# Autodesk Inventor assembly: ThrusterAssembly
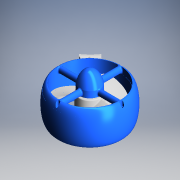
[picture p0: Inventor's stored thumbnail of the model, 180x180]
Saved by Autodesk Inventor 2016 (Build 200138000, 138)
## iProperties
Created: 2016-02-28
Part Number: ThrusterAssembly
Document SubType Name: Assembly
Designer: Willis
Author: Willis
## Documents named in this file (7)
- C:\Users\Willis\Desktop\ROV2015\Thruster Beta\ThrusterAssembly.iam
- C:\Users\Willis\Desktop\ROV2015\Thruster Beta\Body.ipt
- C:\Users\Willis\Desktop\ROV2015\Thruster Beta\Cap.ipt
- C:\Users\Willis\Desktop\ROV2015\Thruster Beta\BrushlessInner.ipt
- C:\Users\Willis\Desktop\ROV2015\Thruster Beta\BrushlessOuter.ipt
- C:\Users\Willis\Desktop\ROV2015\Thruster Beta\Prop_Mk2.ipt
- C:\Users\Willis\Desktop\ROV2015\Thruster Beta\Mount.ipt
## Components (6 placed, 6 different names)
1. Body:1 — Mate:1, Mate:2, Mate:3, Mate:4, Mate:5, Mate:12, Mate:13, Mate:14, Flush:1, Mate:15
2. Cap:1 — Mate:1, Mate:2, Mate:12
3. BrushlessInner:1 — Mate:3, Mate:4, Mate:5, Mate:7, Mate:8, Mate:13
4. BrushlessOuter:1 — Mate:7, Mate:8, Mate:9, Mate:10, Mate:11
5. Prop_Mk2:1 — Mate:9, Mate:10, Mate:11
6. Mount:1 — Mate:14, Flush:1, Mate:15
## Relationships (15: Mate 14, Flush 1)
- Mate:1: Body:1 ↔ Cap:1
- Mate:2: Body:1 ↔ Cap:1
- Mate:3: Body:1 ↔ BrushlessInner:1
- Mate:4: Body:1 ↔ BrushlessInner:1
- Mate:5: Body:1 ↔ BrushlessInner:1
- Mate:7: BrushlessInner:1 ↔ BrushlessOuter:1
- Mate:8 (0.5 mm): BrushlessInner:1 ↔ BrushlessOuter:1
- Mate:9: BrushlessOuter:1 ↔ Prop_Mk2:1
- Mate:10: BrushlessOuter:1 ↔ Prop_Mk2:1
- Mate:11: BrushlessOuter:1 ↔ Prop_Mk2:1
- Mate:12: Body:1 ↔ Cap:1
- Mate:13: Body:1 ↔ BrushlessInner:1
- Mate:14: Body:1 ↔ Mount:1
- Flush:1: Body:1 ↔ Mount:1
- Mate:15: Body:1 ↔ Mount:1
